# Autodesk Inventor assembly: wheel_dual
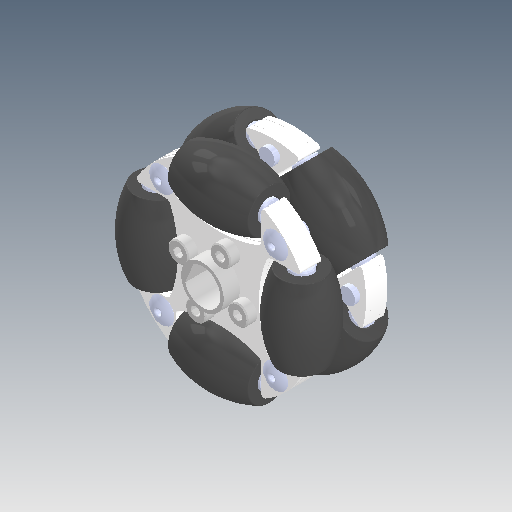
[picture p0: Inventor's stored thumbnail of the model, 512x512]
Saved by Autodesk Inventor 2020 (Build 240168000, 168)
## iProperties
Created: 2019-11-04
Part Number: wheel_dual
Document SubType Name: Assembly
Designer: ball
Author: ball
## Documents named in this file (5)
- C:\FTC\FTC8863CAD\2019 Robot\Odoemetry module\wheel_dual.iam
- C:\FTC\FTC8863CAD\2019 Robot\Odoemetry module\wheel single.iam
- C:\FTC\FTC8863CAD\2019 Robot\Odoemetry module\Our omiwheelinsert.ipt
- C:\FTC\FTC8863CAD\2019 Robot\Odoemetry module\91292A031_TYPE 18-8 SS SOCKET HEAD CAP SCREW.ipt
- C:\FTC\FTC8863CAD\2019 Robot\Odoemetry module\93625A101_TYPE 18-8 M2 STAINLESS STL NYLON-INSERT LOCKNUT.ipt
## Components (11 placed, 4 different names)
1. wheel single:1 [sub-assembly] — Mate:1, Mate:2, Mate:3, Mate:5, Mate:7, Mate:8, Mate:9, Mate:10, Mate:16, Mate:17, Mate:18
2. wheel single:2 [sub-assembly] — Mate:4, Mate:5, Mate:6, Mate:12, Mate:14, Mate:15, Mate:21, Mate:22
3. Our omiwheelinsert:1 — Mate:1, Mate:2, Mate:3, Mate:4, Mate:6
4. 91292A031_TYPE 18-8 SS SOCKET HEAD CAP SCREW:1 — Mate:9, Mate:10, Mate:13
5. 91292A031_TYPE 18-8 SS SOCKET HEAD CAP SCREW:2 — Mate:17, Mate:18, Mate:20
6. 91292A031_TYPE 18-8 SS SOCKET HEAD CAP SCREW:3 — Mate:15, Mate:16, Mate:19
7. 91292A031_TYPE 18-8 SS SOCKET HEAD CAP SCREW:4 — Mate:7, Mate:8, Mate:11
8. 93625A101_TYPE 18-8 M2 STAINLESS STL NYLON-INSERT LOCKNUT:1 — Mate:11, Mate:12
9. 93625A101_TYPE 18-8 M2 STAINLESS STL NYLON-INSERT LOCKNUT:2 — Mate:20, Mate:22
10. 93625A101_TYPE 18-8 M2 STAINLESS STL NYLON-INSERT LOCKNUT:3 — Mate:19, Mate:21
11. 93625A101_TYPE 18-8 M2 STAINLESS STL NYLON-INSERT LOCKNUT:4 — Mate:13, Mate:14
## Relationships (22: Mate 22)
- Mate:1: wheel single:1 ↔ Our omiwheelinsert:1
- Mate:2: wheel single:1 ↔ Our omiwheelinsert:1
- Mate:3: wheel single:1 ↔ Our omiwheelinsert:1
- Mate:4: wheel single:2 ↔ Our omiwheelinsert:1
- Mate:5: wheel single:1 ↔ wheel single:2
- Mate:6: wheel single:2 ↔ Our omiwheelinsert:1
- Mate:7: wheel single:1 ↔ 91292A031_TYPE 18-8 SS SOCKET HEAD CAP SCREW:4
- Mate:8: wheel single:1 ↔ 91292A031_TYPE 18-8 SS SOCKET HEAD CAP SCREW:4
- Mate:9: wheel single:1 ↔ 91292A031_TYPE 18-8 SS SOCKET HEAD CAP SCREW:1
- Mate:10: wheel single:1 ↔ 91292A031_TYPE 18-8 SS SOCKET HEAD CAP SCREW:1
- Mate:11: 91292A031_TYPE 18-8 SS SOCKET HEAD CAP SCREW:4 ↔ 93625A101_TYPE 18-8 M2 STAINLESS STL NYLON-INSERT LOCKNUT:1
- Mate:12: wheel single:2 ↔ 93625A101_TYPE 18-8 M2 STAINLESS STL NYLON-INSERT LOCKNUT:1
- Mate:13: 91292A031_TYPE 18-8 SS SOCKET HEAD CAP SCREW:1 ↔ 93625A101_TYPE 18-8 M2 STAINLESS STL NYLON-INSERT LOCKNUT:4
- Mate:14: wheel single:2 ↔ 93625A101_TYPE 18-8 M2 STAINLESS STL NYLON-INSERT LOCKNUT:4
- Mate:15: wheel single:2 ↔ 91292A031_TYPE 18-8 SS SOCKET HEAD CAP SCREW:3
- Mate:16: wheel single:1 ↔ 91292A031_TYPE 18-8 SS SOCKET HEAD CAP SCREW:3
- Mate:17: wheel single:1 ↔ 91292A031_TYPE 18-8 SS SOCKET HEAD CAP SCREW:2
- Mate:18: wheel single:1 ↔ 91292A031_TYPE 18-8 SS SOCKET HEAD CAP SCREW:2
- Mate:19: 91292A031_TYPE 18-8 SS SOCKET HEAD CAP SCREW:3 ↔ 93625A101_TYPE 18-8 M2 STAINLESS STL NYLON-INSERT LOCKNUT:3
- Mate:20: 91292A031_TYPE 18-8 SS SOCKET HEAD CAP SCREW:2 ↔ 93625A101_TYPE 18-8 M2 STAINLESS STL NYLON-INSERT LOCKNUT:2
- Mate:21: wheel single:2 ↔ 93625A101_TYPE 18-8 M2 STAINLESS STL NYLON-INSERT LOCKNUT:3
- Mate:22: wheel single:2 ↔ 93625A101_TYPE 18-8 M2 STAINLESS STL NYLON-INSERT LOCKNUT:2
